# Autodesk Inventor assembly: новая каретка
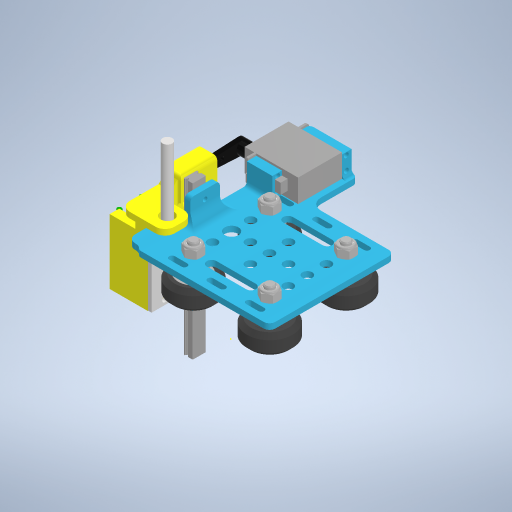
[picture p0: Inventor's stored thumbnail of the model, 512x512]
Saved by Autodesk Inventor 2024.2 (Build 282272000, 272)
## iProperties
Created: 2026-01-31
Part Number: новая каретка
Document SubType Name: Assembly
Designer: katya_notebook
Author: katya_notebook
## iProperties of the stored document V-Slot Gantry Kit - 20mm.iam
Created: 2019-10-15
Part Number: V-Slot Gantry Kit - 20mm
Document SubType Name: Assembly
Designer: katya_notebook
Sending System: Autodesk Translation Framework v8.6.0.1094
Preprocessor: ST-DEVELOPER v18
Title: /Users/ayahni/Desktop/V-Slot Gantry Kit - 20mm.step
## iProperties of the stored document V-Slot Gantry Plate 20mm v1.ipt
Created: 2026-01-31
Part Number: V-Slot Gantry Plate 20mm
Material: SolidWorks Materials|6061-T6 (SS)
Document SubType Name: Modeling
Designer: katya_notebook
Density: 2.7 g/cm^3
Appearance: По умолчанию
Author: katya_notebook
## iProperties of the stored document Ball Bearing 5 x 16 x 5 v1.ipt
Created: 2026-01-31
Part Number: Ball Bearing 5 x 16 x 5
Material: SolidWorks Materials|Plain Carbon Steel
Document SubType Name: Modeling
Designer: katya_notebook
Density: 7.8 g/cm^3
Appearance: По умолчанию
Author: katya_notebook
## iProperties of the stored document Xtreme Solid V Wheel v1.ipt
Created: 2026-01-31
Part Number: Xtreme Solid V Wheel
Material: SolidWorks Materials|PC High Viscosity
Document SubType Name: Modeling
Designer: katya_notebook
Density: 1.19 g/cm^3
Appearance: По умолчанию
Author: katya_notebook
## iProperties of the stored document Aluminum Spacer 6mm v1.ipt
Created: 2026-01-31
Part Number: Aluminum Spacer 6mm
Material: SolidWorks Materials|6061-T6 (SS)
Document SubType Name: Modeling
Designer: katya_notebook
Density: 2.7 g/cm^3
Appearance: По умолчанию
Author: katya_notebook
## iProperties of the stored document Nylon Insert Lock Nut M5 v1.ipt
Created: 2026-01-31
Part Number: Nylon Insert Lock Nut M5
Material: SolidWorks Materials|Plain Carbon Steel
Document SubType Name: Modeling
Designer: katya_notebook
Density: 7.8 g/cm^3
Appearance: По умолчанию
Author: katya_notebook
## iProperties of the stored document Precision Shim 8 x 5 x 1 v1.ipt
Created: 2026-01-31
Part Number: Precision Shim 8 x 5 x 1
Material: SolidWorks Materials|AISI 304
Document SubType Name: Modeling
Designer: katya_notebook
Density: 8 g/cm^3
Appearance: По умолчанию
Author: katya_notebook
## iProperties of the stored document Eccentric Spacer 6mm v1.ipt
Created: 2026-01-31
Part Number: Eccentric Spacer 6mm v1
Material: SolidWorks Materials|AISI 304
Document SubType Name: Modeling
Designer: katya_notebook
Density: 8 g/cm^3
Appearance: По умолчанию
Author: katya_notebook
## iProperties of the stored document Low Profile Screw M5 v1.ipt
Created: 2026-01-31
Part Number: Low Profile Screw M5 v1
Material: SolidWorks Materials|Plain Carbon Steel
Document SubType Name: Modeling
Designer: katya_notebook
Density: 7.8 g/cm^3
Appearance: По умолчанию
Author: katya_notebook
## Documents named in this file (20)
- D:\alletz\construction\новая каретка.iam
- **D:\alletz\construction\новая каретка.iam*LocalDocs*xAaaaq4caAaaaaaaaAaaaaq5rDa*V-Slot Gantry Kit - 20mm.iam
- D:\alletz\construction\MGN7C каретка\MGN7C каретка.ipt
- D:\alletz\construction\JX Servo PDI-HV2006MG\JX Servo PDI-HV2006MG.ipt
- D:\alletz\construction\MHN7C рельса\MHN7C рельса.ipt
- D:\alletz\construction\держатель магнитов на основе.ipt
- D:\alletz\construction\деталь основа каретки.ipt
- D:\alletz\construction\соединяет крепление с магнитом и рельсу.ipt
- D:\alletz\construction\25T Servo Horn Steering Arm M3.ipt
- D:\alletz\construction\винтик.ipt
- D:\alletz\construction\крепление маркера 18мм.ipt
- **D:\alletz\construction\новая каретка.iam*LocalDocs*xAaaaawaaAaaaaaaaAaaaqv4kIh*V-Slot Gantry Plate 20mm v1.ipt
- **D:\alletz\construction\новая каретка.iam*LocalDocs*xAaaaqwdaAaaaaaaaAaaaak53Xc*Low Profile Screw M5 v1.ipt
- **D:\alletz\construction\новая каретка.iam*LocalDocs*xAaaaqhaaAaaaaaaaAaaaqv2uRb*Nylon Insert Lock Nut M5 v1.ipt
- **D:\alletz\construction\новая каретка.iam*LocalDocs*xAaaaqiaaAaaaaaaaAaaaqp2j2f*Aluminum Spacer 6mm v1.ipt
- **D:\alletz\construction\новая каретка.iam*LocalDocs*xAaaaqicaAaaaaaaaAaaaa4atUg*Eccentric Spacer 6mm v1.ipt
- **D:\alletz\construction\новая каретка.iam*LocalDocs*xAaaaahbaAaaaaaaaAaaaaczlSd*Ball Bearing 5 x 16 x 5 v1.ipt
- **D:\alletz\construction\новая каретка.iam*LocalDocs*xAaaaqjdaAaaaaaaaAaaaagpeVg*Precision Shim 8 x 5 x 1 v1.ipt
- **D:\alletz\construction\новая каретка.iam*LocalDocs*xAaaaq3aaAaaaaaaaAaaaavzcTb*Xtreme Solid V Wheel v1.ipt
- D:\alletz\construction\V-Slot Gantry Kit - 20mm.step
## Components (10 placed, 10 different names)
1. V-Slot Gantry Kit - 20mm:1 [sub-assembly] — Заподлицо:1, Заподлицо:2
2. MGN7C каретка:1 — Совмещение:6, Совмещение:7, Заподлицо:9, Заподлицо:10, С поворотом:2
3. JX Servo PDI-HV2006MG:1 — Совмещение:5, Заподлицо:7, Заподлицо:8, С поворотом:1
4. MHN7C рельса:1 — Заподлицо:1, Совмещение:6, Совмещение:7, Заподлицо:9
5. держатель магнитов на основе:1 — Совмещение:4, Заподлицо:5, Заподлицо:6, Заподлицо:13, Заподлицо:14, Заподлицо:15, Совмещение:8, Заподлицо:16, Совмещение:9
6. деталь основа каретки:1 — Заподлицо:2, Совмещение:5, Заподлицо:7, Заподлицо:8, Заподлицо:13, Цилиндрический:1, Заподлицо:14, Заподлицо:15
7. соединяет крепление с магнитом и рельсу:1 — Совмещение:4, Заподлицо:5, Заподлицо:6, Заподлицо:10, С поворотом:2
8. 25T Servo Horn Steering Arm M3:1 — С поворотом:1
9. винтик:1 — Цилиндрический:1
10. крепление маркера 18мм:1 — Совмещение:8, Заподлицо:16, Совмещение:9
## Relationships (21: Flush 12, Mate 6, RevoluteJoint 2, CylindricalJoint 1)
- Заподлицо:1 [Flush] (29.25 mm): V-Slot Gantry Kit - 20mm:1 ↔ MHN7C рельса:1
- Заподлицо:2 [Flush]: V-Slot Gantry Kit - 20mm:1 ↔ деталь основа каретки:1
- Совмещение:4 [Mate]: держатель магнитов на основе:1 ↔ соединяет крепление с магнитом и рельсу:1
- Заподлицо:5 [Flush]: держатель магнитов на основе:1 ↔ соединяет крепление с магнитом и рельсу:1
- Заподлицо:6 [Flush] (1 mm): держатель магнитов на основе:1 ↔ соединяет крепление с магнитом и рельсу:1
- Совмещение:5 [Mate]: JX Servo PDI-HV2006MG:1 ↔ деталь основа каретки:1
- Заподлицо:7 [Flush] (-6 mm): JX Servo PDI-HV2006MG:1 ↔ деталь основа каретки:1
- Заподлицо:8 [Flush] (-20 mm): JX Servo PDI-HV2006MG:1 ↔ деталь основа каретки:1
- Совмещение:6 [Mate]: MGN7C каретка:1 ↔ MHN7C рельса:1
- Совмещение:7 [Mate]: MGN7C каретка:1 ↔ MHN7C рельса:1
- Заподлицо:9 [Flush] (22 mm): MGN7C каретка:1 ↔ MHN7C рельса:1
- С поворотом:1 [RevoluteJoint]: JX Servo PDI-HV2006MG:1 ↔ 25T Servo Horn Steering Arm M3:1
- Заподлицо:10 [Flush]: MGN7C каретка:1 ↔ соединяет крепление с магнитом и рельсу:1
- С поворотом:2 [RevoluteJoint] (-0.4 mm): MGN7C каретка:1 ↔ соединяет крепление с магнитом и рельсу:1
- Заподлицо:13 [Flush]: держатель магнитов на основе:1 ↔ деталь основа каретки:1
- Цилиндрический:1 [CylindricalJoint]: деталь основа каретки:1 ↔ винтик:1
- Заподлицо:14 [Flush]: держатель магнитов на основе:1 ↔ деталь основа каретки:1
- Заподлицо:15 [Flush] (4 mm): держатель магнитов на основе:1 ↔ деталь основа каретки:1
- Совмещение:8 [Mate]: держатель магнитов на основе:1 ↔ крепление маркера 18мм:1
- Заподлицо:16 [Flush]: держатель магнитов на основе:1 ↔ крепление маркера 18мм:1
- Совмещение:9 [Mate] (0.15 mm): держатель магнитов на основе:1 ↔ крепление маркера 18мм:1
